# Autodesk Inventor assembly: s-assy-guide
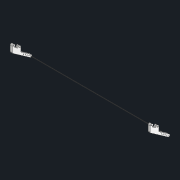
[picture p0: Inventor's stored thumbnail of the model, 180x180]
Saved by Autodesk Inventor 2022 (Build 260153000, 153)
## iProperties
Created: 2021-11-16
Part Number: s-assy-guide
Document SubType Name: Assembly
Designer: Yuta Kage
Author: Yuta Kage
## Documents named in this file (3)
- C:\Users\yuta0\Documents\GitHub\catchrobo_hardware\assy-scara\s-assy-guide.iam
- C:\Users\yuta0\Documents\GitHub\catchrobo_hardware\assy-shooter\shooter_base8[.ipt
- C:\Users\yuta0\Documents\GitHub\catchrobo_hardware\assy-shooter\Part2.ipt
## Components (3 placed, 2 different names)
1. shooter_base8[:1 — メイト:3, メイト:4, フラッシュ:2, メイト:6
2. shooter_base8[:2 — 角度:1, メイト:6
3. Part2:1 — メイト:2, メイト:4, フラッシュ:2, メイト:5
## Relationships (9: Mate 6, Flush 2, Angle 1)
- [Flush]: shooter_base8[:2 ↔ Part2:1
- [Mate]: shooter_base8[:2 ↔ Part2:1
- メイト:2 [Mate]: Part2:1
- メイト:3 [Mate] (303.5 mm): shooter_base8[:1
- メイト:4 [Mate]: shooter_base8[:1 ↔ Part2:1
- フラッシュ:2 [Flush]: shooter_base8[:1 ↔ Part2:1
- メイト:5 [Mate]: Part2:1
- 角度:1 [Angle] (0 deg): shooter_base8[:2
- メイト:6 [Mate]: shooter_base8[:1 ↔ shooter_base8[:2
